# Autodesk Inventor assembly: COMPOSITE_PRINTER_V2
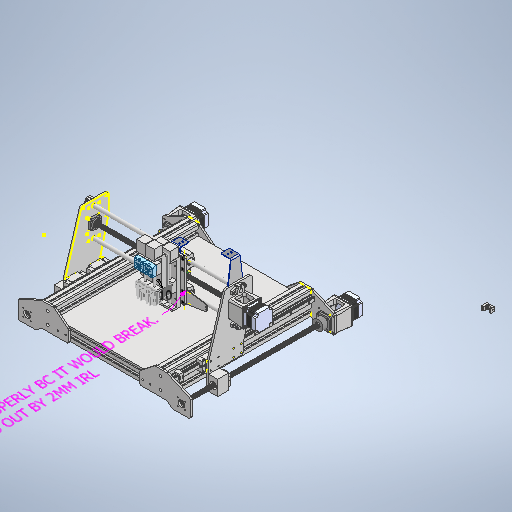
[picture p0: Inventor's stored thumbnail of the model, 512x512]
Saved by Autodesk Inventor 2025.2 (Build 292293000, 293)
## iProperties
Created: 2026-02-05
Part Number: COMPOSITE_PRINTER_V2
Document SubType Name: Assembly
Designer: composite
Author: composite
## Documents named in this file (28)
- H:\01-Members Space\Sam Munro\Extrusion Printer\Printer V2\COMPOSITE_PRINTER_V2.iam
- H:\01-Members Space\Sam Munro\Extrusion Printer\Printer V2\4040_X_BASE.ipt
- H:\01-Members Space\Sam Munro\Extrusion Printer\Printer V2\4080_Y_BASE.ipt
- H:\01-Members Space\Sam Munro\Extrusion Printer\Printer V2\HGR15_Y_RAIL.ipt
- H:\01-Members Space\Sam Munro\Extrusion Printer\Printer V2\hgh15ca_01.ipt
- H:\01-Members Space\Sam Munro\Extrusion Printer\Printer V2\SIDE SUPPORT PLATES.ipt
- H:\01-Members Space\Sam Munro\Extrusion Printer\Printer V2\support_shf12.ipt
- H:\01-Members Space\Sam Munro\Extrusion Printer\Printer V2\178202343-9-stepper_am23hs0420-01\stepper_am23hs0420-01.iam
- H:\01-Members Space\Sam Munro\Extrusion Printer\Printer V2\12MM_X_AXIS_SHAFT.ipt
- H:\01-Members Space\Sam Munro\Extrusion Printer\Printer V2\FF10 Floated Side\FF10 Floated Side\FF10 Floated Side.iam
- H:\01-Members Space\Sam Munro\Extrusion Printer\Printer V2\FK10 Fixed Side - SIMP.ipt
- H:\01-Members Space\Sam Munro\Extrusion Printer\Printer V2\SFU1204-500\SFU1204-500\SFU1204-500.ipt
- H:\01-Members Space\Sam Munro\Extrusion Printer\Printer V2\6.35-8mm COUPLING.ipt
- H:\01-Members Space\Sam Munro\Extrusion Printer\Printer V2\SIDE_SUPPORT_PLATE-PASSIVE.ipt
- H:\01-Members Space\Sam Munro\Extrusion Printer\Printer V2\SCS12UU-DIMP.ipt
- H:\01-Members Space\Sam Munro\Extrusion Printer\Printer V2\SFU1204-3-NUT.ipt
- H:\01-Members Space\Sam Munro\Extrusion Printer\Printer V2\DSG12H - TO_MS_SPEC.ipt
- H:\01-Members Space\Sam Munro\Extrusion Printer\Printer V2\X_PLATE_V2.ipt
- H:\01-Members Space\Sam Munro\Extrusion Printer\Printer V2\6MM_ENDPLATE_FIXEDSIDE.ipt
- H:\01-Members Space\Sam Munro\Extrusion Printer\Printer V2\6MM_ENDPLATE_FLOATINGSIDE.ipt
- H:\01-Members Space\Sam Munro\Extrusion Printer\Printer V2\PRINTESS FILES\SINGLE_SYRINGE_ASSEMBLY.iam
- H:\01-Members Space\Sam Munro\Extrusion Printer\Printer V2\DSG12H ball nut housing\TOOLPLATE.ipt
- H:\01-Members Space\Sam Munro\Extrusion Printer\Printer V2\5537T586_T-Slotted Framing\5537T586_T-Slotted Framing\5537T586_T-Slotted Framing.ipt
- H:\01-Members Space\Sam Munro\Extrusion Printer\Printer V2\XY_MOTOR_MOUNTS_3DP.ipt
- H:\01-Members Space\Sam Munro\Extrusion Printer\Printer V2\HGR_LIMITSWITCHHOLDER.ipt
- H:\01-Members Space\Sam Munro\Extrusion Printer\Printer V2\ENDSTOPPLATE_XAXIS.ipt
- H:\01-Members Space\Sam Munro\Extrusion Printer\Printer V2\DRAGCABLE_XATTACH.ipt
- H:\01-Members Space\Sam Munro\Extrusion Printer\Printer V2\DRAGCABLE_ATTACHMENT.ipt
## Components (63 placed, 27 different names)
1. X_PLATE_V2:1 — Flush:26, Mate:67, Mate:68, Mate:69, Mate:121, Mate:122, Mate:123, Mate:124, Mate:125, Mate:126, Mate:146, Mate:149
2. DSG12H - TO_MS_SPEC:2 — Mate:72, Mate:73, Flush:27, Mate:85, Mate:86
3. 6MM_ENDPLATE_FIXEDSIDE:1 — Flush:28, Flush:29, Mate:74, Flush:30, Mate:75, Mate:76, Mate:77, Mate:78, Mate:79, Mate:80, Mate:81, Mate:90, Mate:91, Mate:138, Mate:139
4. FK10 Fixed Side - SIMP:2 — Mate:76, Mate:77, Mate:78, Mate:82, Mate:83
5. stepper_am23hs0420-01:2 [sub-assembly] — Mate:79, Mate:80, Mate:81, Mate:140
6. SFU1204-500:2 — Mate:82, Mate:83, Mate:84, Mate:120
7. SFU1204-3-NUT:2 — Mate:84, Mate:85, Mate:86
8. 6MM_ENDPLATE_FLOATINGSIDE:1 — Flush:31, Flush:32, Mate:87, Mate:88, Mate:89, Mate:92, Mate:93, Mate:94
9. FF10 Floated Side:2 [sub-assembly] — Mate:87, Mate:88, Mate:89
10. 6MM_ENDPLATE_FIXEDSIDE:2 — Mate:95, Mate:96, Mate:97, Mate:101, Mate:102, Mate:103, Mate:106, Mate:108, Mate:141
11. 6MM_ENDPLATE_FLOATINGSIDE:2 — Mate:98, Mate:99, Mate:100, Mate:117, Mate:119
12. FK10 Fixed Side - SIMP:3 — Mate:101, Mate:102, Mate:103, Mate:104, Mate:105
13. SFU1204-500:3 — Mate:104, Mate:105, Mate:107, Mate:111, Mate:113, Mate:118
14. stepper_am23hs0420-01:3 [sub-assembly] — Mate:106, Mate:107, Mate:108, Mate:116, Mate:142, Mate:143
15. DSG12H - TO_MS_SPEC:3 — Mate:109, Mate:110, Mate:111, Mate:112, Mate:114, Mate:115
16. 6.35-8mm COUPLING:2 — Mate:116
17. 6.35-8mm COUPLING:3 — Mate:120
18. SFU1204-3-NUT:3 — Mate:113, Mate:114, Mate:115
19. FF10 Floated Side:3 [sub-assembly] — Mate:117, Mate:118, Mate:119
20. SINGLE_SYRINGE_ASSEMBLY:1 [sub-assembly] — Mate:121, Mate:122, Mate:123
21. SINGLE_SYRINGE_ASSEMBLY:2 [sub-assembly] — Mate:124, Mate:125, Mate:126
22. TOOLPLATE:1 — Flush:34, Flush:35
23. 5537T586_T-Slotted Framing:2 — Mate:132, Mate:133, Flush:38
24. 5537T586_T-Slotted Framing:4 — Mate:128, Mate:129, Flush:36
25. 5537T586_T-Slotted Framing:7 — Mate:134, Mate:135, Flush:39
26. 5537T586_T-Slotted Framing:8 — Mate:130, Mate:131, Flush:37
27. XY_MOTOR_MOUNTS_3DP:1 — Flush:40, Mate:136, Mate:137
28. XY_MOTOR_MOUNTS_3DP:2 — Mate:138, Mate:139, Mate:140
29. XY_MOTOR_MOUNTS_3DP:3 — Mate:141, Mate:142, Mate:143
30. HGR_LIMITSWITCHHOLDER:1 — Mate:144, Mate:145
31. HGR_LIMITSWITCHHOLDER:2
32. ENDSTOPPLATE_XAXIS:1 — Mate:146, Mate:147, Mate:148
33. DRAGCABLE_XATTACH:1 — Mate:149, Mate:150, Mate:151
34. DRAGCABLE_ATTACHMENT:1 — Flush:41
35. 4040_X_BASE:1 — Flush:1, Flush:2, Flush:3, Mate:1, Flush:4, Flush:5, Mate:2, Flush:6, Flush:31, Flush:32, Flush:34, Mate:131, Mate:132, Flush:38
36. 4040_X_BASE:2 — Flush:1, Flush:2, Flush:7, Flush:28, Flush:29, Flush:35, Mate:128, Flush:36, Mate:135
37. 4080_Y_BASE:1 — Flush:3, Mate:1, Flush:4, Flush:7, Mate:3, Flush:8, Mate:4, Mate:74, Flush:30, Mate:75, Mate:133, Mate:134, Flush:39
38. 4080_Y_BASE:2 — Flush:5, Mate:2, Flush:6, Mate:5, Mate:6, Flush:9, Mate:95, Mate:96, Mate:97, Mate:98, Mate:99, Mate:100, Mate:129, Mate:130, Flush:37
39. HGR15_Y_RAIL:1 — Mate:3, Flush:8, Mate:4, Mate:7, Mate:8, Mate:9, Mate:10, Mate:90, Mate:91, Mate:92, Mate:93, Mate:144, Mate:145
40. HGR15_Y_RAIL:2 — Mate:5, Mate:6, Flush:9, Mate:11, Mate:12, Mate:13, Mate:14
41. hgh15ca_01:1 — Mate:9, Mate:10, Mate:16
42. hgh15ca_01:2 — Mate:7, Mate:8, Mate:16, Flush:10, Flush:12, Mate:19, Mate:127
43. hgh15ca_01:3 — Mate:11, Mate:12, Mate:15, Flush:17, Mate:45
44. hgh15ca_01:4 — Mate:13, Mate:14, Mate:15, Flush:10, Mate:44, Mate:46
45. SIDE SUPPORT PLATES:1 — Flush:12, Mate:17, Mate:18, Mate:19, Mate:20, Mate:21, Mate:22, Mate:23, Mate:24, Mate:25, Angle:1, Mate:30, Angle:2, Mate:36, Mate:57, Angle:3, Mate:70, Mate:72, Mate:73, Flush:27, Flush:33, Mate:94, Mate:127, Flush:40, Flush:41
46. support_shf12:1 — Mate:17, Mate:18, Mate:20, Flush:15, Mate:26
47. support_shf12:4 — Mate:21, Mate:22, Mate:23, Flush:16, Mate:27
48. stepper_am23hs0420-01:1 [sub-assembly] — Mate:24, Mate:25, Angle:1, Mate:136, Mate:137
49. 12MM_X_AXIS_SHAFT:1 — Flush:15, Mate:26, Mate:41, Mate:42, Mate:63, Mate:64
50. 12MM_X_AXIS_SHAFT:2 — Flush:16, Mate:27, Mate:61, Mate:62
51. FF10 Floated Side:1 [sub-assembly] — Mate:39, Mate:40, Mate:43
52. FK10 Fixed Side - SIMP:1 — Mate:30, Angle:2, Mate:32, Mate:33, Mate:36, Angle:3
53. SFU1204-500:1 — Mate:32, Mate:33, Mate:34, Mate:35, Mate:39, Mate:40, Mate:57, Mate:58
54. 6.35-8mm COUPLING:1 — Mate:34, Mate:35
55. SIDE_SUPPORT_PLATE-PASSIVE:1 — Flush:17, Mate:41, Mate:42, Mate:43, Mate:44, Mate:45, Mate:46, Mate:47, Mate:48, Mate:49, Mate:50, Mate:51, Mate:52, Flush:33, Mate:109, Mate:110, Mate:112
56. support_shf12:5 — Mate:50, Mate:51, Mate:52
57. support_shf12:6 — Mate:47, Mate:48, Mate:49
58. SCS12UU-DIMP:1 — Mate:64, Flush:19, Flush:20, Flush:22, Mate:65, Flush:23, Mate:69, Mate:150
59. SCS12UU-DIMP:2 — Mate:63, Flush:20, Flush:21, Mate:65, Flush:24, Flush:25, Mate:151
60. SCS12UU-DIMP:3 — Mate:62, Flush:18, Flush:22, Flush:23, Mate:70, Mate:147
61. SCS12UU-DIMP:4 — Mate:61, Flush:18, Flush:19, Flush:21, Mate:148
62. SFU1204-3-NUT:1 — Mate:58, Mate:59, Mate:60, Mate:66
63. DSG12H - TO_MS_SPEC:1 — Mate:59, Mate:60, Flush:24, Flush:25, Mate:66, Flush:26, Mate:67, Mate:68
## Relationships (182: Mate 141, Flush 38, Angle 3)
- Flush:1: 4040_X_BASE:1 ↔ 4040_X_BASE:2
- Flush:2: 4040_X_BASE:1 ↔ 4040_X_BASE:2
- Flush:3: 4040_X_BASE:1 ↔ 4080_Y_BASE:1
- Mate:1: 4040_X_BASE:1 ↔ 4080_Y_BASE:1
- Flush:4: 4040_X_BASE:1 ↔ 4080_Y_BASE:1
- Flush:5: 4040_X_BASE:1 ↔ 4080_Y_BASE:2
- Mate:2: 4040_X_BASE:1 ↔ 4080_Y_BASE:2
- Flush:6: 4040_X_BASE:1 ↔ 4080_Y_BASE:2
- Flush:7: 4040_X_BASE:2 ↔ 4080_Y_BASE:1
- Mate:3: 4080_Y_BASE:1 ↔ HGR15_Y_RAIL:1
- Flush:8: 4080_Y_BASE:1 ↔ HGR15_Y_RAIL:1
- Mate:4: 4080_Y_BASE:1 ↔ HGR15_Y_RAIL:1
- Mate:5: 4080_Y_BASE:2 ↔ HGR15_Y_RAIL:2
- Mate:6: 4080_Y_BASE:2 ↔ HGR15_Y_RAIL:2
- Flush:9: 4080_Y_BASE:2 ↔ HGR15_Y_RAIL:2
- Mate:7: HGR15_Y_RAIL:1 ↔ hgh15ca_01:2
- Mate:8: HGR15_Y_RAIL:1 ↔ hgh15ca_01:2
- Mate:9: HGR15_Y_RAIL:1 ↔ hgh15ca_01:1
- Mate:10: HGR15_Y_RAIL:1 ↔ hgh15ca_01:1
- Mate:11: HGR15_Y_RAIL:2 ↔ hgh15ca_01:3
- Mate:12: HGR15_Y_RAIL:2 ↔ hgh15ca_01:3
- Mate:13: HGR15_Y_RAIL:2 ↔ hgh15ca_01:4
- Mate:14: HGR15_Y_RAIL:2 ↔ hgh15ca_01:4
- Mate:15 (15 mm): hgh15ca_01:3 ↔ hgh15ca_01:4
- Mate:16 (15 mm): hgh15ca_01:1 ↔ hgh15ca_01:2
- Flush:10: hgh15ca_01:2 ↔ hgh15ca_01:4
- Flush:12: hgh15ca_01:2 ↔ SIDE SUPPORT PLATES:1
- Mate:17: SIDE SUPPORT PLATES:1 ↔ support_shf12:1
- Mate:18: SIDE SUPPORT PLATES:1 ↔ support_shf12:1
- Mate:19: hgh15ca_01:2 ↔ SIDE SUPPORT PLATES:1
- Mate:20: SIDE SUPPORT PLATES:1 ↔ support_shf12:1
- Mate:21: SIDE SUPPORT PLATES:1 ↔ support_shf12:4
- Mate:22: SIDE SUPPORT PLATES:1 ↔ support_shf12:4
- Mate:23: SIDE SUPPORT PLATES:1 ↔ support_shf12:4
- Mate:24 (48 mm): SIDE SUPPORT PLATES:1 ↔ stepper_am23hs0420-01:1
- Mate:25: SIDE SUPPORT PLATES:1 ↔ stepper_am23hs0420-01:1
- Angle:1 (0 deg): SIDE SUPPORT PLATES:1 ↔ stepper_am23hs0420-01:1
- Flush:15: support_shf12:1 ↔ 12MM_X_AXIS_SHAFT:1
- Mate:26: support_shf12:1 ↔ 12MM_X_AXIS_SHAFT:1
- Flush:16: support_shf12:4 ↔ 12MM_X_AXIS_SHAFT:2
- Mate:27: support_shf12:4 ↔ 12MM_X_AXIS_SHAFT:2
- Mate:30: SIDE SUPPORT PLATES:1 ↔ FK10 Fixed Side - SIMP:1
- Angle:2 (0 deg): SIDE SUPPORT PLATES:1 ↔ FK10 Fixed Side - SIMP:1
- Mate:32: FK10 Fixed Side - SIMP:1 ↔ SFU1204-500:1
- Mate:33: FK10 Fixed Side - SIMP:1 ↔ SFU1204-500:1
- Mate:34 (-10 mm): SFU1204-500:1 ↔ 6.35-8mm COUPLING:1
- Mate:35: SFU1204-500:1 ↔ 6.35-8mm COUPLING:1
- Flush:17: hgh15ca_01:3 ↔ SIDE_SUPPORT_PLATE-PASSIVE:1
- Mate:36: SIDE SUPPORT PLATES:1 ↔ FK10 Fixed Side - SIMP:1
- Mate:39: FF10 Floated Side:1 ↔ SFU1204-500:1
- Mate:40: FF10 Floated Side:1 ↔ SFU1204-500:1
- Mate:41: 12MM_X_AXIS_SHAFT:1 ↔ SIDE_SUPPORT_PLATE-PASSIVE:1
- Mate:42: 12MM_X_AXIS_SHAFT:1 ↔ SIDE_SUPPORT_PLATE-PASSIVE:1
- Mate:43: FF10 Floated Side:1 ↔ SIDE_SUPPORT_PLATE-PASSIVE:1
- Mate:44: hgh15ca_01:4 ↔ SIDE_SUPPORT_PLATE-PASSIVE:1
- Mate:45: hgh15ca_01:3 ↔ SIDE_SUPPORT_PLATE-PASSIVE:1
- Mate:46: hgh15ca_01:4 ↔ SIDE_SUPPORT_PLATE-PASSIVE:1
- Mate:47: SIDE_SUPPORT_PLATE-PASSIVE:1 ↔ support_shf12:6
- Mate:48: SIDE_SUPPORT_PLATE-PASSIVE:1 ↔ support_shf12:6
- Mate:49: SIDE_SUPPORT_PLATE-PASSIVE:1 ↔ support_shf12:6
- Mate:50: SIDE_SUPPORT_PLATE-PASSIVE:1 ↔ support_shf12:5
- Mate:51: SIDE_SUPPORT_PLATE-PASSIVE:1 ↔ support_shf12:5
- Mate:52: SIDE_SUPPORT_PLATE-PASSIVE:1 ↔ support_shf12:5
- Mate:57: SIDE SUPPORT PLATES:1 ↔ SFU1204-500:1
- Angle:3 (0 deg): SIDE SUPPORT PLATES:1 ↔ FK10 Fixed Side - SIMP:1
- Mate:58: SFU1204-500:1 ↔ SFU1204-3-NUT:1
- Mate:59: SFU1204-3-NUT:1 ↔ DSG12H - TO_MS_SPEC:1
- Mate:60: SFU1204-3-NUT:1 ↔ DSG12H - TO_MS_SPEC:1
- Mate:61: 12MM_X_AXIS_SHAFT:2 ↔ SCS12UU-DIMP:4
- Mate:62: 12MM_X_AXIS_SHAFT:2 ↔ SCS12UU-DIMP:3
- Mate:63: 12MM_X_AXIS_SHAFT:1 ↔ SCS12UU-DIMP:2
- Mate:64: 12MM_X_AXIS_SHAFT:1 ↔ SCS12UU-DIMP:1
- Flush:18: SCS12UU-DIMP:3 ↔ SCS12UU-DIMP:4
- Flush:19: SCS12UU-DIMP:1 ↔ SCS12UU-DIMP:4
- Flush:20: SCS12UU-DIMP:1 ↔ SCS12UU-DIMP:2
- Flush:21: SCS12UU-DIMP:2 ↔ SCS12UU-DIMP:4
- Flush:22: SCS12UU-DIMP:1 ↔ SCS12UU-DIMP:3
- Mate:65 (10 mm): SCS12UU-DIMP:1 ↔ SCS12UU-DIMP:2
- Flush:23: SCS12UU-DIMP:1 ↔ SCS12UU-DIMP:3
- Flush:24 (23 mm): SCS12UU-DIMP:2 ↔ DSG12H - TO_MS_SPEC:1
- Flush:25: SCS12UU-DIMP:2 ↔ DSG12H - TO_MS_SPEC:1
- Mate:66: SFU1204-3-NUT:1 ↔ DSG12H - TO_MS_SPEC:1
- Flush:26: X_PLATE_V2:1 ↔ DSG12H - TO_MS_SPEC:1
- Mate:67: X_PLATE_V2:1 ↔ DSG12H - TO_MS_SPEC:1
- Mate:68: X_PLATE_V2:1 ↔ DSG12H - TO_MS_SPEC:1
- Mate:69: X_PLATE_V2:1 ↔ SCS12UU-DIMP:1
- Mate:70 (150 mm): SIDE SUPPORT PLATES:1 ↔ SCS12UU-DIMP:3
- Mate:72: DSG12H - TO_MS_SPEC:2 ↔ SIDE SUPPORT PLATES:1
- Mate:73: DSG12H - TO_MS_SPEC:2 ↔ SIDE SUPPORT PLATES:1
- Flush:27: DSG12H - TO_MS_SPEC:2 ↔ SIDE SUPPORT PLATES:1
- Flush:28: 6MM_ENDPLATE_FIXEDSIDE:1 ↔ 4040_X_BASE:2
- Flush:29: 6MM_ENDPLATE_FIXEDSIDE:1 ↔ 4040_X_BASE:2
- Mate:74: 6MM_ENDPLATE_FIXEDSIDE:1 ↔ 4080_Y_BASE:1
- Flush:30: 6MM_ENDPLATE_FIXEDSIDE:1 ↔ 4080_Y_BASE:1
- Mate:75: 6MM_ENDPLATE_FIXEDSIDE:1 ↔ 4080_Y_BASE:1
- Mate:76: 6MM_ENDPLATE_FIXEDSIDE:1 ↔ FK10 Fixed Side - SIMP:2
- Mate:77: 6MM_ENDPLATE_FIXEDSIDE:1 ↔ FK10 Fixed Side - SIMP:2
- Mate:78: 6MM_ENDPLATE_FIXEDSIDE:1 ↔ FK10 Fixed Side - SIMP:2
- Mate:79 (48 mm): 6MM_ENDPLATE_FIXEDSIDE:1 ↔ stepper_am23hs0420-01:2
- Mate:80: 6MM_ENDPLATE_FIXEDSIDE:1 ↔ stepper_am23hs0420-01:2
- Mate:81: 6MM_ENDPLATE_FIXEDSIDE:1 ↔ stepper_am23hs0420-01:2
- Mate:82: FK10 Fixed Side - SIMP:2 ↔ SFU1204-500:2
- Mate:83: FK10 Fixed Side - SIMP:2 ↔ SFU1204-500:2
- Mate:84: SFU1204-500:2 ↔ SFU1204-3-NUT:2
- Mate:85: DSG12H - TO_MS_SPEC:2 ↔ SFU1204-3-NUT:2
- Mate:86: DSG12H - TO_MS_SPEC:2 ↔ SFU1204-3-NUT:2
- Flush:31: 6MM_ENDPLATE_FLOATINGSIDE:1 ↔ 4040_X_BASE:1
- Flush:32: 6MM_ENDPLATE_FLOATINGSIDE:1 ↔ 4040_X_BASE:1
- Mate:87: 6MM_ENDPLATE_FLOATINGSIDE:1 ↔ FF10 Floated Side:2
- Mate:88: 6MM_ENDPLATE_FLOATINGSIDE:1 ↔ FF10 Floated Side:2
- Mate:89: 6MM_ENDPLATE_FLOATINGSIDE:1 ↔ FF10 Floated Side:2
- Mate:90: 6MM_ENDPLATE_FIXEDSIDE:1 ↔ HGR15_Y_RAIL:1
- Mate:91: 6MM_ENDPLATE_FIXEDSIDE:1 ↔ HGR15_Y_RAIL:1
- Mate:92: 6MM_ENDPLATE_FLOATINGSIDE:1 ↔ HGR15_Y_RAIL:1
- Mate:93: 6MM_ENDPLATE_FLOATINGSIDE:1 ↔ HGR15_Y_RAIL:1
- Flush:33: SIDE SUPPORT PLATES:1 ↔ SIDE_SUPPORT_PLATE-PASSIVE:1
- Mate:94 (100 mm): 6MM_ENDPLATE_FLOATINGSIDE:1 ↔ SIDE SUPPORT PLATES:1
- Mate:95: 6MM_ENDPLATE_FIXEDSIDE:2 ↔ 4080_Y_BASE:2
- Mate:96: 6MM_ENDPLATE_FIXEDSIDE:2 ↔ 4080_Y_BASE:2
- Mate:97: 6MM_ENDPLATE_FIXEDSIDE:2 ↔ 4080_Y_BASE:2
- Mate:98: 6MM_ENDPLATE_FLOATINGSIDE:2 ↔ 4080_Y_BASE:2
- Mate:99: 6MM_ENDPLATE_FLOATINGSIDE:2 ↔ 4080_Y_BASE:2
- Mate:100: 6MM_ENDPLATE_FLOATINGSIDE:2 ↔ 4080_Y_BASE:2
- Mate:101: 6MM_ENDPLATE_FIXEDSIDE:2 ↔ FK10 Fixed Side - SIMP:3
- Mate:102: 6MM_ENDPLATE_FIXEDSIDE:2 ↔ FK10 Fixed Side - SIMP:3
- Mate:103: 6MM_ENDPLATE_FIXEDSIDE:2 ↔ FK10 Fixed Side - SIMP:3
- Mate:104: FK10 Fixed Side - SIMP:3 ↔ SFU1204-500:3
- Mate:105: FK10 Fixed Side - SIMP:3 ↔ SFU1204-500:3
- Mate:106 (48 mm): 6MM_ENDPLATE_FIXEDSIDE:2 ↔ stepper_am23hs0420-01:3
- Mate:107: SFU1204-500:3 ↔ stepper_am23hs0420-01:3
- Mate:108: 6MM_ENDPLATE_FIXEDSIDE:2 ↔ stepper_am23hs0420-01:3
- Mate:109: DSG12H - TO_MS_SPEC:3 ↔ SIDE_SUPPORT_PLATE-PASSIVE:1
- Mate:110: DSG12H - TO_MS_SPEC:3 ↔ SIDE_SUPPORT_PLATE-PASSIVE:1
- Mate:111: SFU1204-500:3 ↔ DSG12H - TO_MS_SPEC:3
- Mate:112: DSG12H - TO_MS_SPEC:3 ↔ SIDE_SUPPORT_PLATE-PASSIVE:1
- Mate:113: SFU1204-500:3 ↔ SFU1204-3-NUT:3
- Mate:114: DSG12H - TO_MS_SPEC:3 ↔ SFU1204-3-NUT:3
- Mate:115: DSG12H - TO_MS_SPEC:3 ↔ SFU1204-3-NUT:3
- Mate:116: stepper_am23hs0420-01:3 ↔ 6.35-8mm COUPLING:2
- Mate:117: 6MM_ENDPLATE_FLOATINGSIDE:2 ↔ FF10 Floated Side:3
- Mate:118: SFU1204-500:3 ↔ FF10 Floated Side:3
- Mate:119: 6MM_ENDPLATE_FLOATINGSIDE:2 ↔ FF10 Floated Side:3
- Mate:120: SFU1204-500:2 ↔ 6.35-8mm COUPLING:3
- Mate:121: X_PLATE_V2:1 ↔ SINGLE_SYRINGE_ASSEMBLY:1
- Mate:122: X_PLATE_V2:1 ↔ SINGLE_SYRINGE_ASSEMBLY:1
- Mate:123: X_PLATE_V2:1 ↔ SINGLE_SYRINGE_ASSEMBLY:1
- Mate:124: X_PLATE_V2:1 ↔ SINGLE_SYRINGE_ASSEMBLY:2
- Mate:125: X_PLATE_V2:1 ↔ SINGLE_SYRINGE_ASSEMBLY:2
- Mate:126: X_PLATE_V2:1 ↔ SINGLE_SYRINGE_ASSEMBLY:2
- Flush:34: TOOLPLATE:1 ↔ 4040_X_BASE:1
- Flush:35: TOOLPLATE:1 ↔ 4040_X_BASE:2
- Mate:127: hgh15ca_01:2 ↔ SIDE SUPPORT PLATES:1
- Mate:128: 5537T586_T-Slotted Framing:4 ↔ 4040_X_BASE:2
- Mate:129: 5537T586_T-Slotted Framing:4 ↔ 4080_Y_BASE:2
- Flush:36 (1.75 mm): 5537T586_T-Slotted Framing:4 ↔ 4040_X_BASE:2
- Mate:130: 5537T586_T-Slotted Framing:8 ↔ 4080_Y_BASE:2
- Mate:131: 5537T586_T-Slotted Framing:8 ↔ 4040_X_BASE:1
- Flush:37 (1.75 mm): 5537T586_T-Slotted Framing:8 ↔ 4080_Y_BASE:2
- Mate:132: 5537T586_T-Slotted Framing:2 ↔ 4040_X_BASE:1
- Mate:133: 5537T586_T-Slotted Framing:2 ↔ 4080_Y_BASE:1
- Flush:38 (1.75 mm): 5537T586_T-Slotted Framing:2 ↔ 4040_X_BASE:1
- Mate:134: 5537T586_T-Slotted Framing:7 ↔ 4080_Y_BASE:1
- Mate:135: 5537T586_T-Slotted Framing:7 ↔ 4040_X_BASE:2
- Flush:39 (-1.75 mm): 5537T586_T-Slotted Framing:7 ↔ 4080_Y_BASE:1
- Flush:40: XY_MOTOR_MOUNTS_3DP:1 ↔ SIDE SUPPORT PLATES:1
- Mate:136: XY_MOTOR_MOUNTS_3DP:1 ↔ stepper_am23hs0420-01:1
- Mate:137: XY_MOTOR_MOUNTS_3DP:1 ↔ stepper_am23hs0420-01:1
- Mate:138: 6MM_ENDPLATE_FIXEDSIDE:1 ↔ XY_MOTOR_MOUNTS_3DP:2
- Mate:139: 6MM_ENDPLATE_FIXEDSIDE:1 ↔ XY_MOTOR_MOUNTS_3DP:2
- Mate:140: stepper_am23hs0420-01:2 ↔ XY_MOTOR_MOUNTS_3DP:2
- Mate:141: 6MM_ENDPLATE_FIXEDSIDE:2 ↔ XY_MOTOR_MOUNTS_3DP:3
- Mate:142: stepper_am23hs0420-01:3 ↔ XY_MOTOR_MOUNTS_3DP:3
- Mate:143: stepper_am23hs0420-01:3 ↔ XY_MOTOR_MOUNTS_3DP:3
- Mate:144: HGR_LIMITSWITCHHOLDER:1 ↔ HGR15_Y_RAIL:1
- Mate:145: HGR_LIMITSWITCHHOLDER:1 ↔ HGR15_Y_RAIL:1
- Mate:146: X_PLATE_V2:1 ↔ ENDSTOPPLATE_XAXIS:1
- Mate:147: ENDSTOPPLATE_XAXIS:1 ↔ SCS12UU-DIMP:3
- Mate:148: ENDSTOPPLATE_XAXIS:1 ↔ SCS12UU-DIMP:4
- Mate:149: X_PLATE_V2:1 ↔ DRAGCABLE_XATTACH:1
- Mate:150: DRAGCABLE_XATTACH:1 ↔ SCS12UU-DIMP:1
- Mate:151: DRAGCABLE_XATTACH:1 ↔ SCS12UU-DIMP:2
- Flush:41: DRAGCABLE_ATTACHMENT:1 ↔ SIDE SUPPORT PLATES:1
## Named parameters: X_BASE_LENGTH = 1 mm, CART_SEP = 15 mm, X_MOTOR_STANDOFF = 48 mm, X_CART_SEP = 10 mm
